# Autodesk Inventor assembly: Assembly1
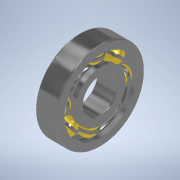
[picture p0: Inventor's stored thumbnail of the model, 180x180]
Saved by Autodesk Inventor 2022.2 (Build 262287030, 287C)
## iProperties
Created: 2022-09-04
Part Number: Assembly1
Document SubType Name: Assembly
Designer: fpopa
Author: fpopa
## Documents named in this file (5)
- C:\Users\fpopa\Desktop\Rulment bile\Assembly1.iam
- C:\Users\fpopa\Desktop\Rulment bile\Outer Ring.ipt
- C:\Users\fpopa\Desktop\Rulment bile\Inner Ring.ipt
- C:\Users\fpopa\Desktop\Rulment bile\Ball.ipt
- C:\Users\fpopa\Desktop\Rulment bile\cage.ipt
## Components (12 placed, 4 different names)
1. Outer Ring:1 — Mate:1, Flush:1, Flush:2
2. Inner Ring:1 — Mate:1, Flush:1, Flush:2, Tangent:1, Mate:3, Mate:5, Mate:9
3. cage:1 — Mate:4, Mate:5, Mate:6, Mate:10
4. cage:2 — Mate:7, Mate:8, Mate:9, Mate:10
5. Ball:1 — Mate:2, Tangent:1, Mate:3, Mate:6
6. Ball:2
7. Ball:3
8. Ball:4
9. Ball:5
10. Ball:6
11. Ball:7
12. Ball:8
## Component patterns: (8 elements, first: Ball:1)
## Relationships (13: Mate 10, Flush 2, Tangent 1)
- Mate:1: Outer Ring:1 ↔ Inner Ring:1
- Flush:1: Outer Ring:1 ↔ Inner Ring:1
- Flush:2: Outer Ring:1 ↔ Inner Ring:1
- Mate:2: Ball:1
- Tangent:1: Inner Ring:1 ↔ Ball:1
- Mate:3: Inner Ring:1 ↔ Ball:1
- Mate:4: cage:1
- Mate:5: Inner Ring:1 ↔ cage:1
- Mate:6: cage:1 ↔ Ball:1
- Mate:7: cage:2
- Mate:8: cage:2
- Mate:9: Inner Ring:1 ↔ cage:2
- Mate:10: cage:1 ↔ cage:2
